# Autodesk Inventor assembly: Assembly2
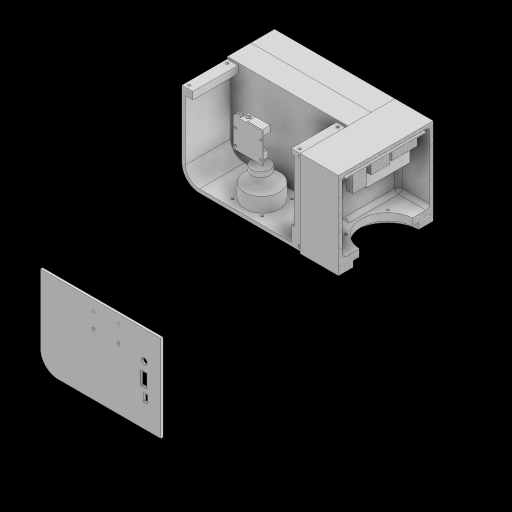
[picture p0: Inventor's stored thumbnail of the model, 512x512]
Saved by Autodesk Inventor 2023 (Build 270158000, 158)
## iProperties
Created: 2022-07-12
Part Number: Assembly2
Document SubType Name: Assembly
Designer: Fuzzyfish
Author: Fuzzyfish
## Documents named in this file (11)
- C:\Users\Fuzzyfish\Documents\Inventor\finalBox\Assembly2.iam
- C:\Users\Fuzzyfish\Documents\Inventor\finalBox\wooferBox.ipt
- C:\Users\Fuzzyfish\Documents\Inventor\finalBox\ElecTweetBox.ipt
- C:\Users\Fuzzyfish\Documents\Inventor\finalBox\3waysplitter.ipt
- C:\Users\Fuzzyfish\Documents\Inventor\finalBox\amp.ipt
- C:\Users\Fuzzyfish\Documents\Inventor\finalBox\tweetwe.ipt
- C:\Users\Fuzzyfish\Documents\Inventor\finalBox\acrylicSidePanel.ipt
- C:\Users\Fuzzyfish\Documents\Inventor\finalBox\acrylicBackPanel.ipt
- C:\Users\Fuzzyfish\Documents\Inventor\finalBox\volumeKnob.ipt
- C:\Users\Fuzzyfish\Documents\Inventor\finalBox\midGroove.ipt
- C:\Users\Fuzzyfish\Documents\Inventor\finalBox\midTongue.ipt
## Components (10 placed, 10 different names)
1. wooferBox:1 — Mate:18, Mate:19, Mate:20, Flush:1, Flush:2, Mate:21, Flush:3, Mate:27, Mate:28, Mate:29
2. ElecTweetBox:1 — Mate:18, Mate:19, Flush:2, Mate:26, Flush:4, Flush:5, Flush:6, Mate:30, Mate:31
3. 3waysplitter:1 — Mate:27, Mate:28, Mate:29
4. amp:1 — Mate:13, Mate:14, Mate:15, Flush:4, Flush:5
5. tweetwe:1 — Flush:6, Mate:30, Mate:31
6. acrylicSidePanel:1
7. acrylicBackPanel:1
8. volumeKnob:1 — Mate:13, Mate:14, Mate:15
9. midGroove:1 — Mate:20, Flush:1, Mate:25
10. midTongue:1 — Mate:21, Flush:3, Mate:25, Mate:26
## Relationships (20: Mate 14, Flush 6)
- Mate:13: amp:1 ↔ volumeKnob:1
- Mate:14: amp:1 ↔ volumeKnob:1
- Mate:15: amp:1 ↔ volumeKnob:1
- Mate:18: wooferBox:1 ↔ ElecTweetBox:1
- Mate:19: wooferBox:1 ↔ ElecTweetBox:1
- Mate:20: wooferBox:1 ↔ midGroove:1
- Flush:1: wooferBox:1 ↔ midGroove:1
- Flush:2: wooferBox:1 ↔ ElecTweetBox:1
- Mate:21: wooferBox:1 ↔ midTongue:1
- Flush:3: wooferBox:1 ↔ midTongue:1
- Mate:25: midGroove:1 ↔ midTongue:1
- Mate:26: ElecTweetBox:1 ↔ midTongue:1
- Flush:4: ElecTweetBox:1 ↔ amp:1
- Flush:5: ElecTweetBox:1 ↔ amp:1
- Mate:27: wooferBox:1 ↔ 3waysplitter:1
- Mate:28: wooferBox:1 ↔ 3waysplitter:1
- Mate:29: wooferBox:1 ↔ 3waysplitter:1
- Flush:6: ElecTweetBox:1 ↔ tweetwe:1
- Mate:30: ElecTweetBox:1 ↔ tweetwe:1
- Mate:31: ElecTweetBox:1 ↔ tweetwe:1
